# Autodesk Inventor assembly: hand_2_1
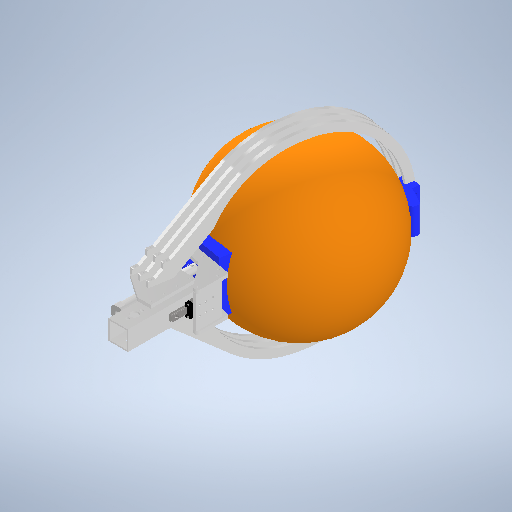
[picture p0: Inventor's stored thumbnail of the model, 512x512]
Saved by Autodesk Inventor 2025.1 (Build 291241000, 241)
## iProperties
Created: 2025-02-02
Part Number: hand_2_1
Document SubType Name: Assembly
Designer: ryogo
Author: ryogo
## Documents named in this file (17)
- D:\A　ロボコン\学ロボ2025\ハンド案②\Workspaces\作業スペース\hand_2_1.iam
- D:\A　ロボコン\学ロボ2025\ハンド案②\Workspaces\作業スペース\hand2_03.ipt
- D:\A　ロボコン\学ロボ2025\ハンド案②\Workspaces\作業スペース\hand2_04.ipt
- D:\A　ロボコン\学ロボ2025\ハンド案②\Workspaces\作業スペース\hand2_05.ipt
- D:\A　ロボコン\学ロボ2025\ハンド案②\Workspaces\作業スペース\hand2_06.ipt
- D:\A　ロボコン\学ロボ2025\ハンド案②\Workspaces\作業スペース\パーツリスト\SSE2B-MX10-455_r.ipt
- D:\A　ロボコン\学ロボ2025\ハンド案②\Workspaces\作業スペース\パーツリスト\SSEB-MX10_b.ipt
- D:\A　ロボコン\学ロボ2025\ハンド案②\Workspaces\作業スペース\hand2_08.ipt
- D:\A　ロボコン\学ロボ2025\ハンド案②\Workspaces\作業スペース\パーツリスト\CJ2B16-15RZ(1_0)_BODY.ipt
- D:\A　ロボコン\学ロボ2025\ハンド案②\Workspaces\作業スペース\パーツリスト\CJ2B16-15Z_ROD.ipt
- D:\A　ロボコン\学ロボ2025\ハンド案②\Workspaces\作業スペース\hand2_09.ipt
- D:\A　ロボコン\学ロボ2025\ハンド案②\Workspaces\作業スペース\hand2_10.ipt
- D:\A　ロボコン\学ロボ2025\ハンド案②\Workspaces\作業スペース\hand2_11.ipt
- D:\A　ロボコン\学ロボ2025\ハンド案②\Workspaces\作業スペース\hand2_12.ipt
- D:\A　ロボコン\学ロボ2025\ハンド案②\Workspaces\作業スペース\バスケボール（仮）.ipt
- D:\A　ロボコン\学ロボ2025\ハンド案②\Workspaces\作業スペース\hand2_13.ipt
- D:\A　ロボコン\学ロボ2025\ハンド案②\Workspaces\作業スペース\hand2_14.ipt
## Components (23 placed, 16 different names)
1. hand2_03:1 — 挿入:17, 挿入:18, フラッシュ:1, フラッシュ:2, 挿入:23, 挿入:40
2. hand2_04:1 — 挿入:11, 挿入:12, 挿入:13, 挿入:14, 挿入:15, 挿入:16, 挿入:25, フラッシュ:3
3. hand2_05:1 — 挿入:5, 挿入:6
4. hand2_06:1 — 挿入:7, 挿入:8
5. hand2_04:2 — 挿入:5, 挿入:6, 挿入:7, 挿入:8, 挿入:9, 挿入:10, 挿入:23, 挿入:26, 挿入:40, フラッシュ:3
6. hand2_05:2 — 挿入:9, 挿入:10, 挿入:42
7. hand2_05:3 — 挿入:11, 挿入:12
8. hand2_05:4 — 挿入:13, 挿入:14, 挿入:41
9. hand2_06:2 — 挿入:15, 挿入:16
10. SSE2B-MX10-455_r:1 — 挿入:17, 挿入:18
11. SSEB-MX10_b:1 — フラッシュ:1, フラッシュ:2, 挿入:33, 挿入:34
12. hand2_08:1 — 挿入:21, 角度:1, 挿入:25, 挿入:26
13. CJ2B16-15RZ(1_0)_BODY:1 — 円柱状:1, 挿入:21, 角度:1
14. CJ2B16-15Z_ROD:1 — 円柱状:1, 挿入:24
15. hand2_09:1 — 挿入:24, 円柱状:2
16. hand2_10:1 — 挿入:29, 挿入:30, 円柱状:2, 挿入:39
17. hand2_11:1 — 挿入:29, 挿入:30, 挿入:31, 挿入:32, 挿入:33, 挿入:34
18. hand2_10:2 — 挿入:31, 挿入:32, 挿入:36, 挿入:37
19. hand2_12:1 — 挿入:36, 挿入:38
20. hand2_12:3 — 挿入:37
21. バスケボール（仮）:1
22. hand2_13:1 — 挿入:38, 挿入:39
23. hand2_14:1 — 挿入:41, 挿入:42
## Relationships (38: Insert 32, Flush 3, CylindricalJoint 2, Angle 1)
- 挿入:5 [Insert]: hand2_05:1 ↔ hand2_04:2
- 挿入:6 [Insert]: hand2_05:1 ↔ hand2_04:2
- 挿入:7 [Insert]: hand2_06:1 ↔ hand2_04:2
- 挿入:8 [Insert]: hand2_06:1 ↔ hand2_04:2
- 挿入:9 [Insert]: hand2_04:2 ↔ hand2_05:2
- 挿入:10 [Insert]: hand2_04:2 ↔ hand2_05:2
- 挿入:11 [Insert]: hand2_04:1 ↔ hand2_05:3
- 挿入:12 [Insert]: hand2_04:1 ↔ hand2_05:3
- 挿入:13 [Insert]: hand2_04:1 ↔ hand2_05:4
- 挿入:14 [Insert]: hand2_04:1 ↔ hand2_05:4
- 挿入:15 [Insert]: hand2_04:1 ↔ hand2_06:2
- 挿入:16 [Insert]: hand2_04:1 ↔ hand2_06:2
- 挿入:17 [Insert]: hand2_03:1 ↔ SSE2B-MX10-455_r:1
- 挿入:18 [Insert]: hand2_03:1 ↔ SSE2B-MX10-455_r:1
- フラッシュ:1 [Flush] (-10 mm): hand2_03:1 ↔ SSEB-MX10_b:1
- フラッシュ:2 [Flush] (-5 mm): hand2_03:1 ↔ SSEB-MX10_b:1
- 円柱状:1 [CylindricalJoint]: CJ2B16-15RZ(1_0)_BODY:1 ↔ CJ2B16-15Z_ROD:1
- 挿入:21 [Insert]: hand2_08:1 ↔ CJ2B16-15RZ(1_0)_BODY:1
- 角度:1 [Angle] (0 deg): hand2_08:1 ↔ CJ2B16-15RZ(1_0)_BODY:1
- 挿入:23 [Insert]: hand2_03:1 ↔ hand2_04:2
- 挿入:24 [Insert] (5 mm): CJ2B16-15Z_ROD:1 ↔ hand2_09:1
- 挿入:25 [Insert]: hand2_04:1 ↔ hand2_08:1
- 挿入:26 [Insert]: hand2_04:2 ↔ hand2_08:1
- 挿入:29 [Insert]: hand2_10:1 ↔ hand2_11:1
- 挿入:30 [Insert]: hand2_10:1 ↔ hand2_11:1
- 挿入:31 [Insert]: hand2_11:1 ↔ hand2_10:2
- 挿入:32 [Insert]: hand2_11:1 ↔ hand2_10:2
- 円柱状:2 [CylindricalJoint]: hand2_09:1 ↔ hand2_10:1
- 挿入:33 [Insert]: SSEB-MX10_b:1 ↔ hand2_11:1
- 挿入:34 [Insert]: SSEB-MX10_b:1 ↔ hand2_11:1
- 挿入:36 [Insert]: hand2_10:2 ↔ hand2_12:1
- 挿入:37 [Insert]: hand2_10:2 ↔ hand2_12:3
- 挿入:38 [Insert]: hand2_12:1 ↔ hand2_13:1
- 挿入:39 [Insert]: hand2_10:1 ↔ hand2_13:1
- 挿入:40 [Insert]: hand2_03:1 ↔ hand2_04:2
- フラッシュ:3 [Flush]: hand2_04:1 ↔ hand2_04:2
- 挿入:41 [Insert]: hand2_05:4 ↔ hand2_14:1
- 挿入:42 [Insert]: hand2_05:2 ↔ hand2_14:1
